# Autodesk Inventor assembly: Stepper Motor
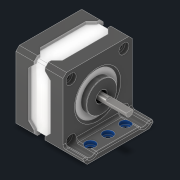
[picture p0: Inventor's stored thumbnail of the model, 180x180]
Saved by Autodesk Inventor 2021.1 (Build 251245000, 245)
## iProperties
Created: 2020-12-15
Part Number: Stepper Motor
Document SubType Name: Assembly
Designer: bestm
Author: bestm
## Documents named in this file (3)
- C:\Users\bestm\McMaster University\Mcdonald, Colin - Course Delivery\4-Projects\P3\Project 3 Autodesk Inventor Files\Updated Files\Stepper Motor\Stepper Motor.iam
- C:\Users\bestm\McMaster University\Mcdonald, Colin - Course Delivery\4-Projects\P3\Project 3 Autodesk Inventor Files\Updated Files\Stepper Motor\Stepper Motor Housing.ipt
- C:\Users\bestm\McMaster University\Mcdonald, Colin - Course Delivery\4-Projects\P3\Project 3 Autodesk Inventor Files\Updated Files\Stepper Motor\Stepper Motor Axle.ipt
## Components (2 placed, 2 different names)
1. Stepper Motor Housing:1 — Mate:1, Mate:2
2. Stepper Motor Axle:1 — Mate:1, Mate:2
## Relationships (2: Mate 2)
- Mate:1: Stepper Motor Housing:1 ↔ Stepper Motor Axle:1
- Mate:2: Stepper Motor Housing:1 ↔ Stepper Motor Axle:1
